# Autodesk Inventor assembly: TS_V1_Fallmagazin_Schieber
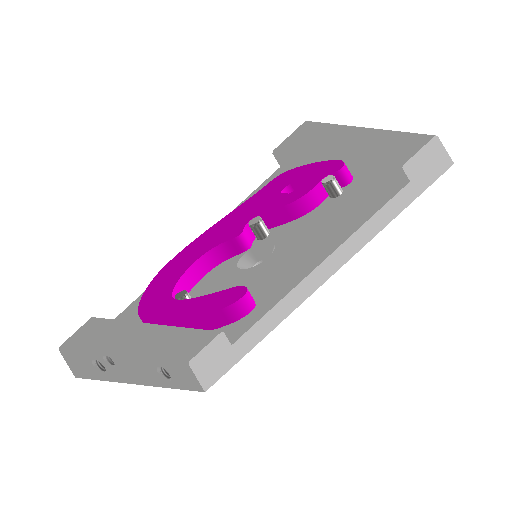
[picture p0: Inventor's stored thumbnail of the model, 512x512]
Saved by Autodesk Inventor 2025.1 (Build 291241000, 241)
## iProperties
Created: 2025-06-11
Part Number: TS_V1_Fallmagazin_Schieber
Document SubType Name: Assembly
Designer: tino
Mass: 52.7362 g
Surface Area: 239.749 cm^2
Volume: 50.6524 cm^3
Density: 1.04114 g/cm^3
Author: tino
## Documents named in this file (5)
- C:\Users\Erik\Erik\Hochschule\3. Semester\CAD\CAD-Paspa\Useless Box\Eigene Bauteile\Fallmagazin\TS_V1_Fallmagazin_Schieber.iam
- C:\Users\Erik\Erik\Hochschule\3. Semester\CAD\CAD-Paspa\Useless Box\Eigene Bauteile\Fallmagazin\TS_V1_Fallmagazin_Schieber_int.ipt
- C:\Users\Erik\Erik\Hochschule\3. Semester\CAD\CAD-Paspa\Useless Box\_Useless_Box\Finger.ipt
- C:\Users\Erik\Erik\Hochschule\3. Semester\CAD\CAD-Paspa\Useless Box\Kaufteile\WUERTH_federndes_Druckstueck\Wuerth_5099201004_Federndes_Druckstueck,_Kugel,_Edelstahl_LOD_High\Wuerth_5099201004_Federndes_Druckstueck,_Kugel,_.iam
- C:\Users\Erik\Erik\Hochschule\3. Semester\CAD\CAD-Paspa\Useless Box\Standart Bauteile\ISO 2338 - 4 m6 x 8.ipt
## Components (7 placed, 4 different names)
1. TS_V1_Fallmagazin_Schieber_int:1 — Passend:3, Passend:4, Passend:5, Passend:6, Passend:7, Passend:8, Passend:9, Passend:10, Passend:11
2. Finger:1 — Passend:3
3. Wuerth_5099201004_Federndes_Druckstueck,_Kugel,_:1 [sub-assembly] — Passend:5
4. Wuerth_5099201004_Federndes_Druckstueck,_Kugel,_:2 [sub-assembly] — Passend:4
5. ISO 2338 4 m6 x 8:1 — Passend:7, Passend:10
6. ISO 2338 4 m6 x 8:2 — Passend:8, Passend:11
7. ISO 2338 4 m6 x 8:3 — Passend:6, Passend:9
## Relationships (9: Mate 9)
- Passend:3 [Mate]: TS_V1_Fallmagazin_Schieber_int:1 ↔ Finger:1
- Passend:4 [Mate]: TS_V1_Fallmagazin_Schieber_int:1 ↔ Wuerth_5099201004_Federndes_Druckstueck,_Kugel,_:2
- Passend:5 [Mate]: TS_V1_Fallmagazin_Schieber_int:1 ↔ Wuerth_5099201004_Federndes_Druckstueck,_Kugel,_:1
- Passend:6 [Mate]: TS_V1_Fallmagazin_Schieber_int:1 ↔ ISO 2338 4 m6 x 8:3
- Passend:7 [Mate]: TS_V1_Fallmagazin_Schieber_int:1 ↔ ISO 2338 4 m6 x 8:1
- Passend:8 [Mate]: TS_V1_Fallmagazin_Schieber_int:1 ↔ ISO 2338 4 m6 x 8:2
- Passend:9 [Mate]: TS_V1_Fallmagazin_Schieber_int:1 ↔ ISO 2338 4 m6 x 8:3
- Passend:10 [Mate]: TS_V1_Fallmagazin_Schieber_int:1 ↔ ISO 2338 4 m6 x 8:1
- Passend:11 [Mate]: TS_V1_Fallmagazin_Schieber_int:1 ↔ ISO 2338 4 m6 x 8:2
